# Autodesk Inventor assembly: panTiltSystemRB04funky
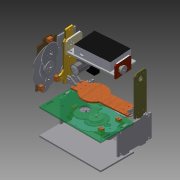
[picture p0: Inventor's stored thumbnail of the model, 180x180]
Saved by Autodesk Inventor 2013 (Build 170138000, 138)
## iProperties
Created: 2014-06-24
Part Number: panTiltSystemRB04funky
Document SubType Name: Assembly
Designer: Nano
Author: Nano
## Documents named in this file (16)
- C:\Users\Nano\Documents\InventorByron\InventorMasterProject\panTiltSystem\panTiltSystemRB04funky.iam
- C:\Users\Nano\Documents\InventorByron\InventorMasterProject\panTiltSystem\baseBoxShortSideRB01.ipt
- C:\Users\Nano\Documents\InventorByron\InventorMasterProject\panTiltSystem\panStepperMountRB01.ipt
- C:\Users\Nano\Documents\InventorByron\InventorMasterProject\panTiltSystem\tiltStructureCrossBeamRB01.ipt
- C:\Users\Nano\Documents\InventorByron\InventorMasterProject\panTiltSystem\tiltColumnStepperSide02_RB01.ipt
- C:\Users\Nano\Documents\InventorByron\InventorMasterProject\panTiltSystem\tiltColumnNonStepperSide02_RB01.ipt
- C:\Users\Nano\Documents\InventorByron\InventorMasterProject\panTiltSystem\projectorMountSide_RB01.ipt
- C:\Users\Nano\Documents\InventorByron\InventorMasterProject\panTiltSystem\projectorMountingBase_RB01.ipt
- C:\Users\Nano\Documents\InventorByron\InventorMasterProject\panTiltSystem\projectorMountOppositeSide_RB01.ipt
- C:\Users\Nano\Documents\InventorByron\InventorMasterProject\panTiltSystem\rotatingSupportShaft_RB01.ipt
- C:\Users\Nano\Documents\InventorByron\InventorMasterProject\panTiltSystem\shaftEndPlate_RB01.ipt
- C:\Users\Nano\Documents\InventorByron\InventorMasterProject\panTiltSystem\aaxaProjector01_RB01.ipt
- C:\Users\Nano\Documents\InventorByron\InventorMasterProject\panTiltSystem\cornerBraceV01.ipt
- C:\Users\Nano\Documents\InventorByron\InventorMasterProject\panTiltSystem\stepperGearBoxSystem.iam
- C:\Users\Nano\Documents\InventorByron\InventorMasterProject\panTiltSystem\dragonfly2CameraAndLens.iam
- C:\Users\Nano\Documents\InventorByron\InventorMasterProject\octoBoto\octoBotoCutFiles\bottomPanel01.ipt
## Components (21 placed, 15 different names)
1. baseBoxShortSideRB01:1 — Mate:76, Mate:77
2. baseBoxShortSideRB01:2
3. panStepperMountRB01:1 — Mate:7
4. tiltStructureCrossBeamRB01:1 — Mate:7, Mate:5, Mate:8, Flush:6, Mate:11, Mate:7, Mate:15, Mate:18, Mate:21, Mate:24, Mate:48, Mate:50, Mate:51, Mate:54, Mate:56
5. tiltColumnStepperSide02_RB01:1 — Mate:5, Mate:8, Flush:6, Mate:32, Mate:49, Mate:52, Mate:53, Mate:73, Angle:7
6. tiltColumnNonStepperSide02_RB01:1 — Mate:11, Mate:7, Mate:39, Mate:55, Mate:57, Mate:58, Mate:59
7. cornerBraceV01:1 — Mate:48, Mate:49, Flush:17, Flush:9
8. cornerBraceV01:2 — Mate:51, Mate:52, Flush:18, Flush:10
9. cornerBraceV01:3 — Mate:54, Mate:55, Flush:20
10. cornerBraceV01:4 — Flush:11, Mate:56, Mate:57, Flush:19
11. projectorMountSide_RB01:1 — Mate:32, Mate:36, Flush:14, Mate:37, Angle:1, Angle:2, Flush:15, Flush:16, Mate:74
12. projectorMountingBase_RB01:1 — Flush:13, Mate:36, Flush:14, Mate:37, Angle:1, Mate:38, Mate:46, Angle:3, Mate:47, Mate:75
13. projectorMountOppositeSide_RB01:1 — Mate:38, Angle:2, Flush:15, Flush:16, Mate:44
14. rotatingSupportShaft_RB01:1 — Mate:39, Mate:40, Mate:41, Mate:42, Mate:43
15. shaftEndPlate_RB01:1 — Mate:40, Mate:42, Mate:44
16. shaftEndPlate_RB01:2 — Mate:41, Mate:43
17. aaxaProjector01_RB01:1 — Mate:46, Angle:3, Mate:47
18. stepperGearBoxSystem:1 [sub-assembly]
19. stepperGearBoxSystem:2 [sub-assembly] — Mate:73, Mate:74, Angle:7
20. dragonfly2CameraAndLens:1 [sub-assembly] — Mate:75
21. bottomPanel01:1 — Mate:76, Mate:77
## Relationships (63: Mate 42, Flush 14, Angle 7)
- Mate:7 (1.016 mm): panStepperMountRB01:1 ↔ tiltStructureCrossBeamRB01:1
- Mate:5: tiltStructureCrossBeamRB01:1 ↔ tiltColumnStepperSide02_RB01:1
- Mate:8: tiltStructureCrossBeamRB01:1 ↔ tiltColumnStepperSide02_RB01:1
- Flush:6: tiltStructureCrossBeamRB01:1 ↔ tiltColumnStepperSide02_RB01:1
- Mate:11: tiltStructureCrossBeamRB01:1 ↔ tiltColumnNonStepperSide02_RB01:1
- Mate:7: tiltStructureCrossBeamRB01:1 ↔ tiltColumnNonStepperSide02_RB01:1
- Mate:15: tiltStructureCrossBeamRB01:1
- Flush:9 (-3.175 mm): cornerBraceV01:1
- Mate:18: tiltStructureCrossBeamRB01:1
- Flush:10 (-3.175 mm): cornerBraceV01:2
- Mate:21: tiltStructureCrossBeamRB01:1
- Flush:11 (-3.175 mm): cornerBraceV01:4
- Mate:24: tiltStructureCrossBeamRB01:1
- Flush:13 (1.8542 mm): projectorMountingBase_RB01:1
- Mate:32 (1.016 mm): tiltColumnStepperSide02_RB01:1 ↔ projectorMountSide_RB01:1
- Mate:36: projectorMountSide_RB01:1 ↔ projectorMountingBase_RB01:1
- Flush:14: projectorMountSide_RB01:1 ↔ projectorMountingBase_RB01:1
- Mate:37 (-3.175 mm): projectorMountSide_RB01:1 ↔ projectorMountingBase_RB01:1
- Angle:1 (0 deg): projectorMountSide_RB01:1 ↔ projectorMountingBase_RB01:1
- Mate:38: projectorMountingBase_RB01:1 ↔ projectorMountOppositeSide_RB01:1
- Angle:2 (0 deg): projectorMountSide_RB01:1 ↔ projectorMountOppositeSide_RB01:1
- Flush:15: projectorMountSide_RB01:1 ↔ projectorMountOppositeSide_RB01:1
- Flush:16: projectorMountSide_RB01:1 ↔ projectorMountOppositeSide_RB01:1
- Mate:39: tiltColumnNonStepperSide02_RB01:1 ↔ rotatingSupportShaft_RB01:1
- Mate:40: rotatingSupportShaft_RB01:1 ↔ shaftEndPlate_RB01:1
- Mate:41: rotatingSupportShaft_RB01:1 ↔ shaftEndPlate_RB01:2
- Mate:42: rotatingSupportShaft_RB01:1 ↔ shaftEndPlate_RB01:1
- Mate:43: rotatingSupportShaft_RB01:1 ↔ shaftEndPlate_RB01:2
- Mate:44 (1.016 mm): projectorMountOppositeSide_RB01:1 ↔ shaftEndPlate_RB01:1
- Mate:46: projectorMountingBase_RB01:1 ↔ aaxaProjector01_RB01:1
- Angle:3 (0 deg): projectorMountingBase_RB01:1 ↔ aaxaProjector01_RB01:1
- Mate:47: projectorMountingBase_RB01:1 ↔ aaxaProjector01_RB01:1
- Mate:48: tiltStructureCrossBeamRB01:1 ↔ cornerBraceV01:1
- Mate:49: tiltColumnStepperSide02_RB01:1 ↔ cornerBraceV01:1
- Flush:17 (-3.175 mm): cornerBraceV01:1
- [Angle] (0 deg): tiltColumnNonStepperSide02_RB01:1 ↔ stepperGearBoxSystem:1
- [Angle] (0 deg): projectorMountingBase_RB01:1 ↔ stepperGearBoxSystem:1
- Mate:50: tiltStructureCrossBeamRB01:1
- Mate:51: tiltStructureCrossBeamRB01:1 ↔ cornerBraceV01:2
- Mate:52: tiltColumnStepperSide02_RB01:1 ↔ cornerBraceV01:2
- Flush:18 (-3.175 mm): cornerBraceV01:2
- Mate:53: tiltColumnStepperSide02_RB01:1
- Mate:54: tiltStructureCrossBeamRB01:1 ↔ cornerBraceV01:3
- Mate:55: tiltColumnNonStepperSide02_RB01:1 ↔ cornerBraceV01:3
- Mate:56: tiltStructureCrossBeamRB01:1 ↔ cornerBraceV01:4
- Mate:57: tiltColumnNonStepperSide02_RB01:1 ↔ cornerBraceV01:4
- Flush:19 (-3.175 mm): cornerBraceV01:4
- Flush:20 (-3.175 mm): cornerBraceV01:3
- Mate:58: tiltColumnNonStepperSide02_RB01:1
- Mate:59: tiltColumnNonStepperSide02_RB01:1
- [Mate]: panStepperMountRB01:1 ↔ stepperGearBoxSystem:1
- [Mate] (3.175 mm): panStepperMountRB01:1 ↔ stepperGearBoxSystem:1
- [Angle] (0 deg): panStepperMountRB01:1 ↔ stepperGearBoxSystem:1
- [Mate]: panStepperMountRB01:1 ↔ stepperGearBoxSystem:1
- [Mate]: panStepperMountRB01:1 ↔ stepperGearBoxSystem:1
- [Flush]: panStepperMountRB01:1 ↔ stepperGearBoxSystem:1
- [Flush]: panStepperMountRB01:1 ↔ stepperGearBoxSystem:1
- Mate:73: tiltColumnStepperSide02_RB01:1 ↔ stepperGearBoxSystem:2
- Mate:74: projectorMountSide_RB01:1 ↔ stepperGearBoxSystem:2
- Angle:7 (0 deg): tiltColumnStepperSide02_RB01:1 ↔ stepperGearBoxSystem:2
- Mate:75: projectorMountingBase_RB01:1 ↔ dragonfly2CameraAndLens:1
- Mate:76: baseBoxShortSideRB01:1 ↔ bottomPanel01:1
- Mate:77: baseBoxShortSideRB01:1 ↔ bottomPanel01:1
